# Autodesk Inventor assembly: WheelAssembly
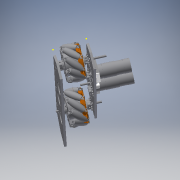
[picture p0: Inventor's stored thumbnail of the model, 180x180]
Saved by Autodesk Inventor 2017 (Build 210142000, 142)
## iProperties
Created: 2016-09-10
Part Number: WheelAssembly
Document SubType Name: Assembly
Designer: RoboticsUser
Author: RoboticsUser
## Documents named in this file (10)
- C:\Robotics\CAD\2016-17_CAD\WheelAssemble2.0 - left.iam
- C:\Robotics\CAD\COTSParts\Actobotics\545 parts\545556.ipt
- C:\Robotics\CAD\COTSParts\Actobotics\615 parts\615102.ipt
- C:\Robotics\CAD\COTSParts\Actobotics\634 parts\634080.ipt
- C:\Robotics\CAD\COTSParts\Motors\Andymark 2964  NeveRest 40 Motor.ipt
- C:\Robotics\CAD\COTSParts\Tetrix\tetrix-motor-mounts-1.snapshot.1\Tetrex 2pc motor mount.ipt
- C:\Robotics\CAD\COTSParts\Actobotics\545 parts\545456.ipt
- C:\Robotics\CAD\COTSParts\Wheels\AndyMark Mecanum Wheels\100mm Aluminum Mecanum wheels.ipt
- C:\Robotics\CAD\2016-17_CAD\DrainTrainPlate2.0.iam
- C:\Robotics\CAD\2016-17_CAD\DriveTrainPlate -Inside.ipt
## Components (24 placed, 9 different names)
1. 545556:2 — Mate:10, Mate:13, Mate:47
2. 615102:4 — Insert:110
3. 634080:2 — Mate:10, Mate:12, Mate:26, Mate:32, Mate:45, Mate:56, Insert:103, Mate:65
4. 545556:6 — Insert:83, Mate:73
5. 634080:3 — Mate:28, Mate:30, Mate:50, Mate:66, Mate:68, Mate:71, Mate:74
6. Andymark 2964  NeveRest 40 Motor:2 — Mate:43, Insert:108, Insert:109
7. 545556:8 — Mate:43, Mate:72
8. 545556:9 — Insert:110
9. Andymark 2964  NeveRest 40 Motor:3 — Insert:111
10. Tetrex 2pc motor mount:1 — Mate:69
11. Tetrex 2pc motor mount:2 — Mate:75, Mate:76
12. 545456:1 — Mate:12, Mate:13, Insert:89
13. 545456:3 — Insert:83, Insert:88
14. 615102:6 — Insert:109, Mate:72
15. 615102:7 — Mate:45, Mate:47, Mate:70
16. 100mm Aluminum Mecanum wheels:1 — Insert:88, Mate:27, Mate:50
17. 100mm Aluminum Mecanum wheels:2 — Insert:89, Mate:25
18. 545456:4 — Mate:25, Mate:26, Mate:31
19. 545456:5 — Mate:27, Mate:28, Mate:29
20. 545556:12 — Mate:29, Mate:30, Mate:54
21. 545556:13 — Mate:31, Mate:32, Mate:59
22. DrainTrainPlate2.0:1 [sub-assembly] — Mate:54, Mate:56, Mate:59, Mate:65, Mate:66, Mate:68
23. DriveTrainPlate -Inside:1 — Insert:103, Mate:69, Mate:70, Insert:108, Mate:71, Mate:75, Mate:76, Insert:111
24. 615102:8 — Mate:73, Mate:74
## Relationships (37: Mate 29, Insert 8)
- Insert:83: 545556:6 ↔ 545456:3
- Mate:10: 545556:2 ↔ 634080:2
- Mate:12: 634080:2 ↔ 545456:1
- Mate:13: 545556:2 ↔ 545456:1
- Insert:88: 545456:3 ↔ 100mm Aluminum Mecanum wheels:1
- Insert:89: 545456:1 ↔ 100mm Aluminum Mecanum wheels:2
- Mate:25: 100mm Aluminum Mecanum wheels:2 ↔ 545456:4
- Mate:26: 634080:2 ↔ 545456:4
- Mate:27: 100mm Aluminum Mecanum wheels:1 ↔ 545456:5
- Mate:28: 634080:3 ↔ 545456:5
- Mate:29: 545456:5 ↔ 545556:12
- Mate:30: 634080:3 ↔ 545556:12
- Mate:31: 545456:4 ↔ 545556:13
- Mate:32: 634080:2 ↔ 545556:13
- Mate:43: Andymark 2964  NeveRest 40 Motor:2 ↔ 545556:8
- Mate:45: 634080:2 ↔ 615102:7
- Mate:47: 545556:2 ↔ 615102:7
- Mate:50: 634080:3 ↔ 100mm Aluminum Mecanum wheels:1
- Mate:54: 545556:12 ↔ DrainTrainPlate2.0:1
- Mate:56: 634080:2 ↔ DrainTrainPlate2.0:1
- Mate:59: 545556:13 ↔ DrainTrainPlate2.0:1
- Insert:103 (36.0426 mm): 634080:2 ↔ DriveTrainPlate -Inside:1
- Mate:65 (-6.35 mm): 634080:2 ↔ DrainTrainPlate2.0:1
- Mate:66 (-6.35 mm): 634080:3 ↔ DrainTrainPlate2.0:1
- Mate:68: 634080:3 ↔ DrainTrainPlate2.0:1
- Mate:69: Tetrex 2pc motor mount:1 ↔ DriveTrainPlate -Inside:1
- Mate:70 (3.175 mm): 615102:7 ↔ DriveTrainPlate -Inside:1
- Insert:108: Andymark 2964  NeveRest 40 Motor:2 ↔ DriveTrainPlate -Inside:1
- Mate:71 (6.35 mm): 634080:3 ↔ DriveTrainPlate -Inside:1
- Insert:109 (-6.35 mm): Andymark 2964  NeveRest 40 Motor:2 ↔ 615102:6
- Mate:72: 545556:8 ↔ 615102:6
- Mate:73: 545556:6 ↔ 615102:8
- Mate:74: 634080:3 ↔ 615102:8
- Mate:75: Tetrex 2pc motor mount:2 ↔ DriveTrainPlate -Inside:1
- Mate:76: Tetrex 2pc motor mount:2 ↔ DriveTrainPlate -Inside:1
- Insert:110: 615102:4 ↔ 545556:9
- Insert:111 (25.4 mm): Andymark 2964  NeveRest 40 Motor:3 ↔ DriveTrainPlate -Inside:1
